# Autodesk Inventor assembly: sborka
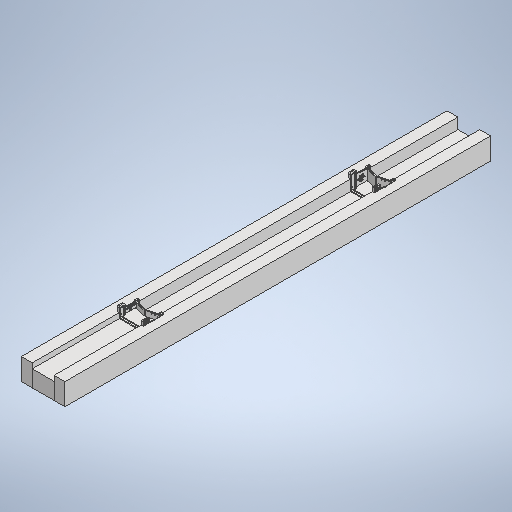
[picture p0: Inventor's stored thumbnail of the model, 512x512]
Saved by Autodesk Inventor 2025.2 (Build 292293000, 293)
## iProperties
Created: 2025-01-19
Part Number: sborka
Document SubType Name: Assembly
Designer: Admin
Author: Admin
## Documents named in this file (11)
- D:\YandexDisk\YandexDisk\2024-2025\Предпроф\shluz\sborka.iam
- D:\YandexDisk\YandexDisk\2024-2025\Предпроф\shluz\bottom_bief.ipt
- D:\YandexDisk\YandexDisk\2024-2025\Предпроф\shluz\only_gate.ipt
- D:\YandexDisk\YandexDisk\2024-2025\Предпроф\shluz\only_gate_MIR.ipt
- D:\YandexDisk\YandexDisk\2024-2025\Предпроф\shluz\only_top_gate.ipt
- D:\YandexDisk\YandexDisk\2024-2025\Предпроф\shluz\top_bief.ipt
- D:\YandexDisk\YandexDisk\2024-2025\Предпроф\shluz\only_top_gate_MIR.ipt
- D:\YandexDisk\YandexDisk\2024-2025\Предпроф\shluz\ground_all.ipt
- D:\YandexDisk\YandexDisk\2024-2025\Предпроф\shluz\side_panel.ipt
- D:\YandexDisk\YandexDisk\2024-2025\Предпроф\shluz\side_panel_MIR.ipt
- D:\YandexDisk\YandexDisk\2024-2025\Предпроф\shluz\STL\gates_top_holder.ipt
## Components (13 placed, 10 different names)
1. bottom_bief:1 — Вставка:1, Вставка:2, Заподлицо:1, Заподлицо:2, Совмещение:1, Заподлицо:9, Вставка:5, Вставка:6, Вставка:7
2. only_gate:1 — Вставка:1
3. only_gate_MIR:1 — Вставка:2, Совмещение:7
4. only_top_gate:1 — Вставка:3
5. top_bief:1 — Вставка:3, Вставка:4, Заподлицо:1, Заподлицо:2, Совмещение:1, Совмещение:2, Совмещение:3, Заподлицо:3, Вставка:8, Вставка:9, Вставка:10
6. only_top_gate_MIR:1 — Вставка:4, Совмещение:8
7. ground_all:1 — Совмещение:2, Совмещение:3, Заподлицо:3, Заподлицо:4, Заподлицо:6, Совмещение:5, Совмещение:6, Заподлицо:7, Заподлицо:8
8. side_panel:1 — Заподлицо:4, Заподлицо:6, Совмещение:5
9. side_panel_MIR:1 — Совмещение:6, Заподлицо:7, Заподлицо:8
10. gates_top_holder:1 — Заподлицо:9, Вставка:7, Совмещение:7
11. gates_top_holder:2 — Вставка:8, Совмещение:8
12. gates_top_holder:3 — Вставка:5, Вставка:6
13. gates_top_holder:4 — Вставка:9, Вставка:10
## Relationships (25: Insert 10, Flush 8, Mate 7)
- Вставка:1 [Insert] (0.5 mm): bottom_bief:1 ↔ only_gate:1
- Вставка:2 [Insert] (0.5 mm): bottom_bief:1 ↔ only_gate_MIR:1
- Вставка:3 [Insert] (0.5 mm): only_top_gate:1 ↔ top_bief:1
- Вставка:4 [Insert] (0.5 mm): top_bief:1 ↔ only_top_gate_MIR:1
- Заподлицо:1 [Flush]: bottom_bief:1 ↔ top_bief:1
- Заподлицо:2 [Flush]: bottom_bief:1 ↔ top_bief:1
- Совмещение:1 [Mate] (970 mm): bottom_bief:1 ↔ top_bief:1
- Совмещение:2 [Mate]: top_bief:1 ↔ ground_all:1
- Совмещение:3 [Mate]: top_bief:1 ↔ ground_all:1
- Заподлицо:3 [Flush] (10 mm): top_bief:1 ↔ ground_all:1
- Заподлицо:4 [Flush]: ground_all:1 ↔ side_panel:1
- Заподлицо:6 [Flush]: ground_all:1 ↔ side_panel:1
- Совмещение:5 [Mate]: ground_all:1 ↔ side_panel:1
- Совмещение:6 [Mate]: ground_all:1 ↔ side_panel_MIR:1
- Заподлицо:7 [Flush]: ground_all:1 ↔ side_panel_MIR:1
- Заподлицо:8 [Flush]: ground_all:1 ↔ side_panel_MIR:1
- Заподлицо:9 [Flush]: bottom_bief:1 ↔ gates_top_holder:1
- Вставка:5 [Insert]: bottom_bief:1 ↔ gates_top_holder:3
- Вставка:6 [Insert]: bottom_bief:1 ↔ gates_top_holder:3
- Вставка:7 [Insert]: bottom_bief:1 ↔ gates_top_holder:1
- Совмещение:7 [Mate]: only_gate_MIR:1 ↔ gates_top_holder:1
- Вставка:8 [Insert]: top_bief:1 ↔ gates_top_holder:2
- Совмещение:8 [Mate]: only_top_gate_MIR:1 ↔ gates_top_holder:2
- Вставка:9 [Insert]: top_bief:1 ↔ gates_top_holder:4
- Вставка:10 [Insert]: top_bief:1 ↔ gates_top_holder:4
